# Autodesk Inventor assembly: Flywheel shit
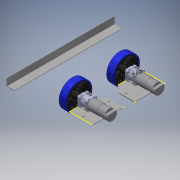
[picture p0: Inventor's stored thumbnail of the model, 180x180]
Saved by Autodesk Inventor 2017 (Build 210142000, 142)
## iProperties
Created: 2016-10-15
Part Number: Flywheel shit
Document SubType Name: Assembly
Designer: Aditya
Author: Aditya
## Documents named in this file (5)
- C:\Users\Aditya\Documents\GitHub\RobotuxCAD\Team Robotux 15-16 Robot Cad Assets\Flywheel shit.iam
- C:\Users\Aditya\Documents\GitHub\RobotuxCAD\Team Robotux 15-16 Robot Cad Assets\Flywheel Headpiece.ipt
- C:\Users\Aditya\Documents\GitHub\RobotuxCAD\Team Robotux 15-16 Robot Cad Assets\Flywheel w motor.iam
- C:\Users\Aditya\Documents\GitHub\RobotuxCAD\Team Robotux 15-16 Robot Cad Assets\Flywheel Motor Plate.ipt
- C:\Users\Aditya\Documents\GitHub\RobotuxCAD\Team Robotux 15-16 Robot Cad Assets\Flywheel Motor Plate_MIR.ipt
## Components (5 placed, 4 different names)
1. Flywheel Headpiece:1
2. Flywheel w motor:1 [sub-assembly] — Mate:1, Flush:1, Mate:2
3. Flywheel Motor Plate:1 — Mate:1, Flush:1, Mate:2
4. Flywheel Motor Plate_MIR:1 — Mate:3, Mate:4, Mate:5
5. Flywheel w motor:2 [sub-assembly] — Mate:3, Mate:4, Mate:5
## Relationships (6: Mate 5, Flush 1)
- Mate:1: Flywheel w motor:1 ↔ Flywheel Motor Plate:1
- Flush:1: Flywheel w motor:1 ↔ Flywheel Motor Plate:1
- Mate:2: Flywheel w motor:1 ↔ Flywheel Motor Plate:1
- Mate:3: Flywheel Motor Plate_MIR:1 ↔ Flywheel w motor:2
- Mate:4: Flywheel Motor Plate_MIR:1 ↔ Flywheel w motor:2
- Mate:5: Flywheel Motor Plate_MIR:1 ↔ Flywheel w motor:2
